# Autodesk Inventor assembly: PEC12R-4017F-N0024
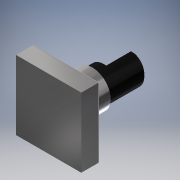
[picture p0: Inventor's stored thumbnail of the model, 180x180]
Saved by Autodesk Inventor 2018 (Build 220112000, 112)
## iProperties
Created: 2018-01-11
Part Number: PEC12R-4017F-N0024
Document SubType Name: Assembly
Designer: Moochster
Author: Moochster
## Documents named in this file (3)
- C:\Users\Moochster\OneDrive\Documents\2018 UBC\ELEC 391\Controller\CAD\PEC12R-4017F-N0024.iam
- C:\Users\Moochster\OneDrive\Documents\2018 UBC\ELEC 391\Controller\CAD\PEC12R-4017F-N0024 Base.ipt
- C:\Users\Moochster\OneDrive\Documents\2018 UBC\ELEC 391\Controller\CAD\PEC12R-4017F-N0024 Shaft.ipt
## Components (2 placed, 2 different names)
1. PEC12R-4017F-N0024 Base:1 — Mate:1, Mate:2
2. PEC12R-4017F-N0024 Shaft:1 — Mate:1, Mate:2
## Relationships (2: Mate 2)
- Mate:1: PEC12R-4017F-N0024 Base:1 ↔ PEC12R-4017F-N0024 Shaft:1
- Mate:2: PEC12R-4017F-N0024 Base:1 ↔ PEC12R-4017F-N0024 Shaft:1
